# Autodesk Inventor assembly: test-model-SPG27
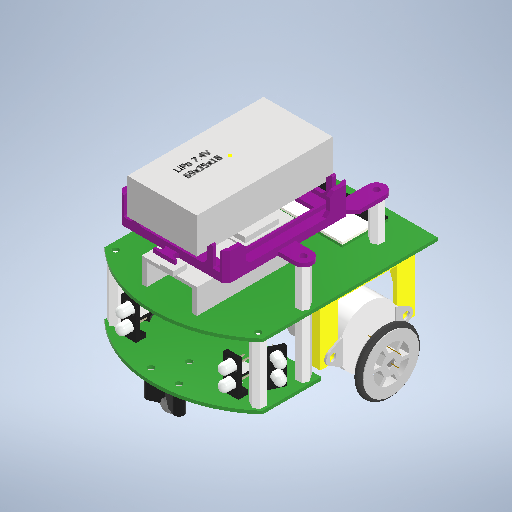
[picture p0: Inventor's stored thumbnail of the model, 512x512]
Saved by Autodesk Inventor 2025.3 (Build 293356030, 356C)
## iProperties
Created: 2025-08-17
Part Number: test-model-SPG27
Document SubType Name: Assembly
Designer: daisuke
Author: daisuke
## Documents named in this file (15)
- G:\マイドライブ\project\micro-mouse\3D-Model\test-model-SPG27-W30.iam
- G:\マイドライブ\project\micro-mouse\3D-Model\BaseBoard-SPG27.ipt
- G:\マイドライブ\project\micro-mouse\3D-Model\SPG27_asm.iam
- G:\マイドライブ\project\micro-mouse\3D-Model\SensorBoard-SPG27.ipt
- G:\マイドライブ\project\micro-mouse\3D-Model\BallCaster-H16.ipt
- G:\マイドライブ\project\micro-mouse\3D-Model\Ground.ipt
- G:\マイドライブ\project\micro-mouse\3D-Model\ESP32-DevKitC.ipt
- G:\マイドライブ\project\micro-mouse\3D-Model\Photo-Sensor.iam
- G:\マイドライブ\project\micro-mouse\3D-Model\AQM1602Y.ipt
- G:\マイドライブ\project\micro-mouse\3D-Model\LiPo-7.4V-69x35x18.ipt
- G:\マイドライブ\project\micro-mouse\3D-Model\Battery-Holder-SPG27-1x4-A.ipt
- G:\マイドライブ\project\micro-mouse\3D-Model\Wheel-D30C.ipt
- G:\マイドライブ\project\micro-mouse\3D-Model\O-ring_D31.ipt
- G:\マイドライブ\project\micro-mouse\3D-Model\Spacer-M3H30.ipt
- G:\マイドライブ\project\micro-mouse\3D-Model\Spacer-M3H20.ipt
## Components (26 placed, 14 different names)
1. BaseBoard-SPG27:1 — メイト:15, メイト:20, メイト:40, メイト:41, メイト:42, メイト:43, メイト:44, メイト:45, メイト:46, メイト:47, メイト:51, メイト:52, メイト:53, メイト:54, メイト:55, メイト:56, メイト:61, メイト:62, メイト:63, メイト:64, メイト:66, メイト:67, メイト:68, メイト:72
2. SensorBoard-SPG27:1 — メイト:9, メイト:10, メイト:11, メイト:16, メイト:17, メイト:18, メイト:19, メイト:48, メイト:49, メイト:50, 角度:1
3. BallCaster-H16:1 — メイト:9, メイト:10, メイト:11
4. Ground:1 — 角度:1
5. ESP32-DevKitC:1 — メイト:15
6. Photo-Sensor:1 [sub-assembly] — メイト:17
7. Photo-Sensor:2 [sub-assembly] — メイト:18
8. Photo-Sensor:3 [sub-assembly] — メイト:16
9. Photo-Sensor:4 [sub-assembly] — メイト:19
10. AQM1602Y:1 — メイト:20
11. LiPo-7.4V-69x35x18:1
12. Battery-Holder-SPG27-1x4-A:1 — メイト:69, メイト:70, メイト:71
13. Wheel-D30C:1 — メイト:57, フラッシュ:1, メイト:60
14. Wheel-D30C:2 — メイト:58, フラッシュ:2, メイト:59
15. O-ring_D31:1 — メイト:60
16. O-ring_D31:2 — メイト:59
17. Spacer-M3H30:1 — メイト:40, メイト:41, メイト:48
18. Spacer-M3H30:2 — メイト:44, メイト:47, メイト:49, メイト:50
19. Spacer-M3H30:3 — メイト:42, メイト:43
20. Spacer-M3H30:4 — メイト:45, メイト:46
21. SPG27_asm:1 [sub-assembly] — メイト:51, メイト:52, メイト:53, メイト:57, フラッシュ:1
22. SPG27_asm:2 [sub-assembly] — メイト:54, メイト:55, メイト:56, メイト:58, フラッシュ:2
23. Spacer-M3H20:1 — メイト:61, メイト:63
24. Spacer-M3H20:2 — メイト:62, メイト:64, メイト:69
25. Spacer-M3H20:3 — メイト:67, メイト:68, メイト:70, メイト:71
26. Spacer-M3H20:4 — メイト:66, メイト:72
## Relationships (44: Mate 41, Flush 2, Angle 1)
- メイト:9 [Mate]: SensorBoard-SPG27:1 ↔ BallCaster-H16:1
- メイト:10 [Mate]: SensorBoard-SPG27:1 ↔ BallCaster-H16:1
- メイト:11 [Mate]: SensorBoard-SPG27:1 ↔ BallCaster-H16:1
- メイト:15 [Mate]: BaseBoard-SPG27:1 ↔ ESP32-DevKitC:1
- メイト:16 [Mate]: SensorBoard-SPG27:1 ↔ Photo-Sensor:3
- メイト:17 [Mate]: SensorBoard-SPG27:1 ↔ Photo-Sensor:1
- メイト:18 [Mate]: SensorBoard-SPG27:1 ↔ Photo-Sensor:2
- メイト:19 [Mate]: SensorBoard-SPG27:1 ↔ Photo-Sensor:4
- メイト:20 [Mate]: BaseBoard-SPG27:1 ↔ AQM1602Y:1
- メイト:40 [Mate]: BaseBoard-SPG27:1 ↔ Spacer-M3H30:1
- メイト:41 [Mate]: BaseBoard-SPG27:1 ↔ Spacer-M3H30:1
- メイト:42 [Mate]: BaseBoard-SPG27:1 ↔ Spacer-M3H30:3
- メイト:43 [Mate]: BaseBoard-SPG27:1 ↔ Spacer-M3H30:3
- メイト:44 [Mate]: BaseBoard-SPG27:1 ↔ Spacer-M3H30:2
- メイト:45 [Mate]: BaseBoard-SPG27:1 ↔ Spacer-M3H30:4
- メイト:46 [Mate]: BaseBoard-SPG27:1 ↔ Spacer-M3H30:4
- メイト:47 [Mate]: BaseBoard-SPG27:1 ↔ Spacer-M3H30:2
- メイト:48 [Mate]: SensorBoard-SPG27:1 ↔ Spacer-M3H30:1
- メイト:49 [Mate]: SensorBoard-SPG27:1 ↔ Spacer-M3H30:2
- メイト:50 [Mate]: SensorBoard-SPG27:1 ↔ Spacer-M3H30:2
- メイト:51 [Mate]: BaseBoard-SPG27:1 ↔ SPG27_asm:1
- メイト:52 [Mate]: BaseBoard-SPG27:1 ↔ SPG27_asm:1
- メイト:53 [Mate]: BaseBoard-SPG27:1 ↔ SPG27_asm:1
- メイト:54 [Mate]: BaseBoard-SPG27:1 ↔ SPG27_asm:2
- メイト:55 [Mate]: BaseBoard-SPG27:1 ↔ SPG27_asm:2
- メイト:56 [Mate]: BaseBoard-SPG27:1 ↔ SPG27_asm:2
- メイト:57 [Mate]: Wheel-D30C:1 ↔ SPG27_asm:1
- フラッシュ:1 [Flush]: Wheel-D30C:1 ↔ SPG27_asm:1
- メイト:58 [Mate]: Wheel-D30C:2 ↔ SPG27_asm:2
- フラッシュ:2 [Flush]: Wheel-D30C:2 ↔ SPG27_asm:2
- メイト:59 [Mate]: Wheel-D30C:2 ↔ O-ring_D31:2
- メイト:60 [Mate]: Wheel-D30C:1 ↔ O-ring_D31:1
- 角度:1 [Angle] (0 deg): SensorBoard-SPG27:1 ↔ Ground:1
- メイト:61 [Mate]: BaseBoard-SPG27:1 ↔ Spacer-M3H20:1
- メイト:62 [Mate]: BaseBoard-SPG27:1 ↔ Spacer-M3H20:2
- メイト:63 [Mate]: BaseBoard-SPG27:1 ↔ Spacer-M3H20:1
- メイト:64 [Mate]: BaseBoard-SPG27:1 ↔ Spacer-M3H20:2
- メイト:66 [Mate]: BaseBoard-SPG27:1 ↔ Spacer-M3H20:4
- メイト:67 [Mate]: BaseBoard-SPG27:1 ↔ Spacer-M3H20:3
- メイト:68 [Mate]: BaseBoard-SPG27:1 ↔ Spacer-M3H20:3
- メイト:69 [Mate]: Battery-Holder-SPG27-1x4-A:1 ↔ Spacer-M3H20:2
- メイト:70 [Mate]: Battery-Holder-SPG27-1x4-A:1 ↔ Spacer-M3H20:3
- メイト:71 [Mate]: Battery-Holder-SPG27-1x4-A:1 ↔ Spacer-M3H20:3
- メイト:72 [Mate]: BaseBoard-SPG27:1 ↔ Spacer-M3H20:4
